# Autodesk Inventor assembly: TruckWithWheels
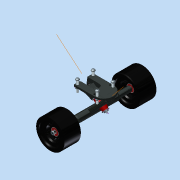
[picture p0: Inventor's stored thumbnail of the model, 180x180]
Saved by Autodesk Inventor 2015 (Build 190159000, 159)
## iProperties
Created: 2015-11-06
Part Number: TruckWithWheels
Document SubType Name: Assembly
Designer: Raphael
Author: Raphael
## Documents named in this file (3)
- \\psf\Home\Documents\electric-skateboard\CAD\TruckWithWheels.iam
- \\psf\Home\Documents\electric-skateboard\CAD\ParisTruck.iam
- \\psf\Home\Documents\electric-skateboard\CAD\WheelWithBearing.iam
## Components (3 placed, 2 different names)
1. ParisTruck:1 [sub-assembly] — Mate:1, Mate:2, Mate:4, Mate:5
2. WheelWithBearing:1 [sub-assembly] — Mate:1, Mate:5
3. WheelWithBearing:2 [sub-assembly] — Mate:2, Mate:4
## Relationships (4: Mate 4)
- Mate:1: ParisTruck:1 ↔ WheelWithBearing:1
- Mate:2: ParisTruck:1 ↔ WheelWithBearing:2
- Mate:4 (1 mm): ParisTruck:1 ↔ WheelWithBearing:2
- Mate:5 (1 mm): ParisTruck:1 ↔ WheelWithBearing:1
